# Autodesk Inventor assembly: deep focus adapter
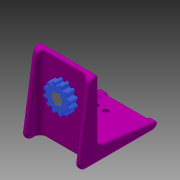
[picture p0: Inventor's stored thumbnail of the model, 180x180]
Saved by Autodesk Inventor 2015 SP2 (Build 190223200, 223)
## iProperties
Created: 2015-05-21
Part Number: deep focus adapter
Document SubType Name: Assembly
Designer: caleb
Author: caleb
## Documents named in this file (4)
- C:\cygwin64\home\caleb\3d\designs\deep-focus-scanning-adapter\deep focus adapter.iam
- C:\cygwin64\home\caleb\3d\designs\deep-focus-scanning-adapter\macro scanner.ipt
- C:\cygwin64\home\caleb\3d\designs\deep-focus-scanning-adapter\knurled nut.ipt
- C:\Users\caleb\Documents\Inventor\Content Center Files\R2015\en-US\ANSI ASME B18.2.1(2)\ANSI_ASME B18.2.1 - 1_4-20 UNC - 0.5(2).ipt
## Components (3 placed, 3 different names)
1. macro scanner:1 — Mate:1, Mate:2, Flush:1, Flush:2, Flush:3
2. knurled nut:1 — Mate:1, Mate:2, Mate:3, Mate:4
3. Hex Bolt - Inch 1/4-20 UNC - 0.5:1 — Mate:3, Mate:4
## Relationships (7: Mate 4, Flush 3)
- Mate:1: macro scanner:1 ↔ knurled nut:1
- Mate:2: macro scanner:1 ↔ knurled nut:1
- Mate:3: knurled nut:1 ↔ Hex Bolt - Inch 1/4-20 UNC - 0.5:1
- Mate:4: knurled nut:1 ↔ Hex Bolt - Inch 1/4-20 UNC - 0.5:1
- Flush:1: macro scanner:1
- Flush:2: macro scanner:1
- Flush:3: macro scanner:1
